# Autodesk Inventor assembly: VR Button Box assembly
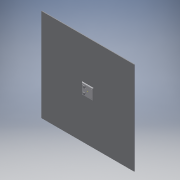
[picture p0: Inventor's stored thumbnail of the model, 180x180]
Saved by Autodesk Inventor 2018 (Build 220112000, 112)
## iProperties
Created: 2019-10-17
Part Number: VR Button Box assembly
Document SubType Name: Assembly
Designer: Jacob
Author: Jacob
## Documents named in this file (7)
- C:\Users\Jacob\git_repos\POE-AIO\CAD Files\VR CAD Files\VR Button Box assembly.iam
- C:\Users\Jacob\git_repos\POE-AIO\CAD Files\2 gang light switch plate.ipt
- C:\Users\Jacob\git_repos\POE-AIO\CAD Files\VR CAD Files\More Accurate Button.ipt
- C:\Users\Jacob\git_repos\POE-AIO\CAD Files\VR CAD Files\More Accurate Button Square.ipt
- C:\Users\Jacob\git_repos\POE-AIO\CAD Files\Screw for button box.ipt
- C:\Users\Jacob\git_repos\POE-AIO\CAD Files\Button box back part.ipt
- C:\Users\Jacob\git_repos\POE-AIO\CAD Files\New Parts\Wall.ipt
## Components (11 placed, 6 different names)
1. 2 gang light switch plate:1 — Mate:10, Mate:11, Mate:12, Mate:13, Mate:14, Mate:15, Mate:22, Mate:23, Mate:24, Mate:25, Mate:26, Mate:27, Mate:28, Mate:29, Mate:32, Mate:33, Mate:34
2. More Accurate Button:1 — Mate:10, Mate:11, Mate:12, Mate:16, Mate:17, Mate:18
3. More Accurate Button:2 — Mate:13, Mate:14, Mate:15, Mate:19, Mate:20, Mate:21
4. More Accurate Button Square:1 — Mate:19, Mate:20, Mate:21
5. More Accurate Button Square:2 — Mate:16, Mate:17, Mate:18
6. Screw for button box:1 — Mate:25, Mate:27
7. Screw for button box:2 — Mate:22, Mate:28
8. Screw for button box:3 — Mate:23, Mate:26
9. Screw for button box:4 — Mate:24, Mate:29
10. Button box back part:1 — Mate:30, Flush:1, Mate:31, Mate:32, Mate:33
11. Wall:1 — Mate:30, Flush:1, Mate:31, Mate:34
## Relationships (26: Mate 25, Flush 1)
- Mate:10: 2 gang light switch plate:1 ↔ More Accurate Button:1
- Mate:11: 2 gang light switch plate:1 ↔ More Accurate Button:1
- Mate:12: 2 gang light switch plate:1 ↔ More Accurate Button:1
- Mate:13: 2 gang light switch plate:1 ↔ More Accurate Button:2
- Mate:14: 2 gang light switch plate:1 ↔ More Accurate Button:2
- Mate:15: 2 gang light switch plate:1 ↔ More Accurate Button:2
- Mate:16: More Accurate Button:1 ↔ More Accurate Button Square:2
- Mate:17: More Accurate Button:1 ↔ More Accurate Button Square:2
- Mate:18: More Accurate Button:1 ↔ More Accurate Button Square:2
- Mate:19: More Accurate Button:2 ↔ More Accurate Button Square:1
- Mate:20: More Accurate Button:2 ↔ More Accurate Button Square:1
- Mate:21: More Accurate Button:2 ↔ More Accurate Button Square:1
- Mate:22: 2 gang light switch plate:1 ↔ Screw for button box:2
- Mate:23: 2 gang light switch plate:1 ↔ Screw for button box:3
- Mate:24: 2 gang light switch plate:1 ↔ Screw for button box:4
- Mate:25: 2 gang light switch plate:1 ↔ Screw for button box:1
- Mate:26: 2 gang light switch plate:1 ↔ Screw for button box:3
- Mate:27: 2 gang light switch plate:1 ↔ Screw for button box:1
- Mate:28: 2 gang light switch plate:1 ↔ Screw for button box:2
- Mate:29: 2 gang light switch plate:1 ↔ Screw for button box:4
- Mate:30: Button box back part:1 ↔ Wall:1
- Flush:1: Button box back part:1 ↔ Wall:1
- Mate:31: Button box back part:1 ↔ Wall:1
- Mate:32: 2 gang light switch plate:1 ↔ Button box back part:1
- Mate:33: 2 gang light switch plate:1 ↔ Button box back part:1
- Mate:34: 2 gang light switch plate:1 ↔ Wall:1
